# Autodesk Inventor assembly: AM14U4 Square Frame Half
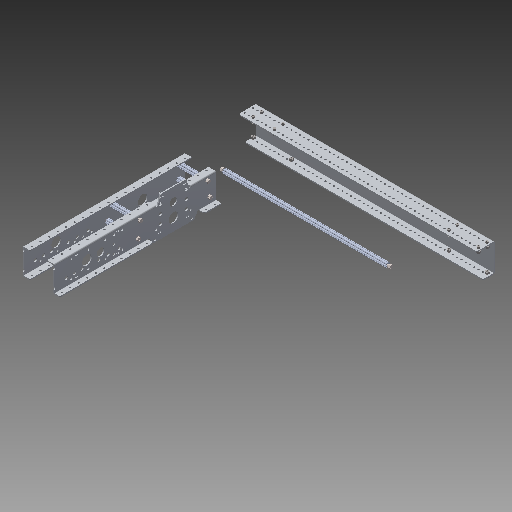
[picture p0: Inventor's stored thumbnail of the model, 512x512]
Saved by Autodesk Inventor 2017 (Build 210142000, 142)
## iProperties
Part Number: AM14U4 Square Frame Half
Material: 一般
Document SubType Name: Assembly
Designer: IJA
Author: IJA
Revision Number: ANY
## Documents named in this file (8)
- D:\Works\Robot2\AM14U4 Square Frame Half.iam
- D:\Works\Robot2\am-xxxx AM14U4 End Plate Square.ipt
- D:\Works\Robot2\am-1002 and am-1042 10-32 x 0500 and Nylock Nut Assembly.iam
- D:\Works\Robot2\FHTS 0.25-20-0.75_FHTS 0.25-20-G-0.75-C.ipt
- D:\Works\Robot2\3.375in Churro.ipt
- D:\Works\Robot2\19.25in Churro.ipt
- D:\Works\Robot2\am-xxxx AM14U4 Outside Plate Square_DefaultSM-FLAT-PATTERN_MIR2.ipt
- D:\Works\Robot2\am-xxxx AM14U4 Inside Plate Square2.ipt
## Components (30 placed, 30 different names)
1. am-xxxx AM14U4 End Plate Square_82 — 貼合:2, 貼合:3
2. am-1002 and am-1042 10-32 x 0500 and Nylock Nut Assembly_85 [sub-assembly] — 貼合:2
3. am-1002 and am-1042 10-32 x 0500 and Nylock Nut Assembly_86 [sub-assembly] — 貼合:3
4. am-1002 and am-1042 10-32 x 0500 and Nylock Nut Assembly_87 [sub-assembly]
5. am-1002 and am-1042 10-32 x 0500 and Nylock Nut Assembly_88 [sub-assembly]
6. am-1002 and am-1042 10-32 x 0500 and Nylock Nut Assembly_89 [sub-assembly]
7. am-1002 and am-1042 10-32 x 0500 and Nylock Nut Assembly_90 [sub-assembly]
8. am-1002 and am-1042 10-32 x 0500 and Nylock Nut Assembly_91 [sub-assembly]
9. am-1002 and am-1042 10-32 x 0500 and Nylock Nut Assembly_92 [sub-assembly]
10. am-1002 and am-1042 10-32 x 0500 and Nylock Nut Assembly_93 [sub-assembly]
11. FHTS 0.25-20-0.75_FHTS 0.25-20-G-0.75-C_94
12. FHTS 0.25-20-0.75_FHTS 0.25-20-G-0.75-C_95
13. FHTS 0.25-20-0.75_FHTS 0.25-20-G-0.75-C_96
14. FHTS 0.25-20-0.75_FHTS 0.25-20-G-0.75-C_97
15. FHTS 0.25-20-0.75_FHTS 0.25-20-G-0.75-C_98
16. FHTS 0.25-20-0.75_FHTS 0.25-20-G-0.75-C_99
17. FHTS 0.25-20-0.75_FHTS 0.25-20-G-0.75-C_100
18. FHTS 0.25-20-0.75_FHTS 0.25-20-G-0.75-C_101
19. 3.375in Churro_102
20. 3.375in Churro_103
21. 3.375in Churro_104
22. 3.375in Churro_105
23. am-1002 and am-1042 10-32 x 0500 and Nylock Nut Assembly_106 [sub-assembly]
24. am-1002 and am-1042 10-32 x 0500 and Nylock Nut Assembly_107 [sub-assembly]
25. am-1002 and am-1042 10-32 x 0500 and Nylock Nut Assembly_108 [sub-assembly]
26. 19.25in Churro_109
27. FHTS 0.25-20-0.75_FHTS 0.25-20-G-0.75-C_110
28. FHTS 0.25-20-0.75_FHTS 0.25-20-G-0.75-C_111
29. am-xxxx AM14U4 Outside Plate Square_DefaultSM-FLAT-PATTERN_MIR2:1
30. am-xxxx AM14U4 Inside Plate Square2:1
## Relationships (2: Mate 2)
- 貼合:2 [Mate]: am-xxxx AM14U4 End Plate Square_82 ↔ am-1002 and am-1042 10-32 x 0500 and Nylock Nut Assembly_85
- 貼合:3 [Mate]: am-xxxx AM14U4 End Plate Square_82 ↔ am-1002 and am-1042 10-32 x 0500 and Nylock Nut Assembly_86
